# Autodesk Inventor assembly: Assembly1
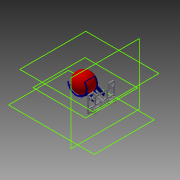
[picture p0: Inventor's stored thumbnail of the model, 180x180]
Saved by Autodesk Inventor 2014 (Build 180170000, 170)
## iProperties
Created: 2014-01-06
Part Number: Assembly1
Document SubType Name: Assembly
Designer: Tristan Debrunner
Author: Tristan Debrunner
## Documents named in this file (17)
- C:\Users\Tristan Debrunner\Documents\FRC 2014\Chassis\Assembly1.iam
- C:\Users\Tristan Debrunner\Documents\FRC 2014\Chassis\32 in bar.ipt
- C:\Users\Tristan Debrunner\Documents\FRC 2014\Chassis\21 in bar.ipt
- C:\Users\Tristan Debrunner\Documents\FRC 2014\Chassis\Corner.ipt
- C:\Users\Tristan Debrunner\Documents\FRC 2014\Chassis\8 in bar.ipt
- C:\Users\Tristan Debrunner\Documents\FRC 2014\Chassis\6 in bar.ipt
- C:\Users\Tristan Debrunner\Documents\FRC 2014\Chassis\Other corner.ipt
- C:\Users\Tristan Debrunner\Documents\FRC 2014\Chassis\2 hole plate.ipt
- C:\Users\Tristan Debrunner\Documents\Inventor\CIMple Box.iam
- C:\Users\Tristan Debrunner\Documents\FRC 2014\Claw Design\Inner.ipt
- C:\Users\Tristan Debrunner\Documents\FRC 2014\Claw Design\rod.ipt
- C:\Users\Tristan Debrunner\Documents\FRC 2014\Claw Design\Outer.ipt
- C:\Users\Tristan Debrunner\Documents\FRC 2014\Chassis\wheel.ipt
- C:\Users\Tristan Debrunner\Documents\FRC 2014\Chassis\Piston.iam
- C:\Users\Tristan Debrunner\Documents\FRC 2014\Chassis\5 in bar.ipt
- C:\Users\Tristan Debrunner\Documents\FRC 2014\Chassis\PG-71-am-0914.ipt
- C:\Users\Tristan Debrunner\Documents\FRC 2014\Chassis\ball.ipt
## Components (57 placed, 16 different names)
1. 32 in bar:1 — Mate:1, Mate:2, Angle:1, Mate:6, Mate:7, Mate:8, Mate:11, Mate:116, Mate:121
2. 21 in bar:1 — Mate:3, Mate:4, Angle:2, Angle:3, Mate:5, Mate:19, Mate:20, Mate:23, Mate:55, Mate:56, Mate:60, Mate:61, Mate:62, Mate:65
3. 21 in bar:2 — Mate:9, Mate:10, Mate:12, Mate:13, Mate:14, Mate:17, Mate:51, Mate:52, Mate:54, Mate:67, Mate:68, Mate:72, Angle:8
4. Corner:1 — Mate:1, Mate:2, Mate:3, Mate:4, Angle:1, Angle:2, Angle:3, Mate:5, Mate:6
5. Corner:2 — Mate:7, Mate:8, Mate:9, Mate:10, Mate:11, Mate:12
6. Corner:3 — Mate:19, Mate:20, Mate:21, Mate:22, Mate:23, Mate:24
7. Corner:4 — Mate:13, Mate:14, Mate:15, Mate:16, Mate:17, Mate:18
8. 6 in bar:1 — Mate:21, Mate:22, Mate:24, Mate:31, Mate:32, Mate:35
9. 6 in bar:2 — Mate:15, Mate:16, Mate:18, Mate:25, Mate:26, Mate:29, Flush:1
10. 6 in bar:3 — Mate:33, Mate:34, Mate:36, Mate:43, Mate:44, Mate:48
11. 6 in bar:4 — Mate:27, Mate:28, Mate:30, Mate:37, Mate:38, Mate:42
12. Corner:5 — Mate:25, Mate:26, Mate:27, Mate:28, Mate:29, Mate:30
13. Corner:6 — Mate:31, Mate:32, Mate:33, Mate:34, Mate:35, Mate:36
14. 32 in bar:2 — Mate:39, Mate:40, Mate:41, Mate:45, Mate:46, Mate:47, Mate:49, Mate:50, Mate:53, Mate:57, Mate:58, Mate:59, Mate:82, Mate:85, Mate:87, Mate:90, Mate:92, Mate:94, Mate:96
15. Corner:7 — Mate:37, Mate:38, Mate:39, Mate:40, Mate:41, Mate:42
16. Corner:8 — Mate:43, Mate:44, Mate:45, Mate:46, Mate:47, Mate:48
17. Corner:9 — Mate:49, Mate:50, Mate:51, Mate:52, Mate:53, Mate:54
18. Corner:10 — Mate:55, Mate:56, Mate:57, Mate:58, Mate:59, Mate:60
19. Corner:11 — Mate:61, Mate:62, Mate:63, Mate:64, Mate:65, Mate:66
20. 32 in bar:3 — Mate:63, Mate:64, Mate:66, Mate:69, Mate:70, Mate:71, Mate:73, Mate:76, Mate:77, Mate:79, Mate:81, Mate:98, Mate:100, Mate:102, Mate:117, Mate:118, Mate:122, Mate:123, Mate:129, Mate:130, Mate:131, Mate:132, Angle:6, Angle:7
21. Corner:12 — Mate:67, Mate:68, Mate:69, Mate:70, Mate:71, Mate:72
22. 8 in bar:1 — Mate:74, Mate:75, Mate:78, Mate:80, Mate:83, Mate:84, Mate:86, Mate:88, Mate:107, Mate:108, Mate:109
23. 8 in bar:2 — Mate:89, Mate:91, Mate:93, Mate:95, Mate:97, Mate:99, Mate:101, Mate:103, Mate:104, Mate:105, Mate:106
24. Other corner:1 — Mate:73, Mate:74, Mate:78
25. Other corner:2 — Mate:75, Mate:76, Mate:77
26. 2 hole plate:1 — Mate:79, Mate:80, Mate:81
27. Other corner:3 — Mate:82, Mate:83
28. Other corner:4 — Mate:84, Mate:85
29. 2 hole plate:2 — Mate:86, Mate:87, Mate:88
30. 2 hole plate:3 — Mate:89, Mate:90, Mate:92
31. 2 hole plate:4 — Mate:91, Mate:98, Mate:103
32. Other corner:5 — Mate:93, Mate:94
33. Other corner:6 — Mate:95, Mate:96, Mate:97
34. Other corner:7 — Mate:101, Mate:102
35. Other corner:8 — Mate:99, Mate:100
36. Corner:13 — Mate:104, Mate:105, Mate:106, Mate:110, Mate:111, Mate:112
37. Corner:14 — Mate:107, Mate:108, Mate:109, Mate:113, Mate:114, Mate:115
38. 8 in bar:3 — Mate:110, Mate:111, Mate:112, Mate:127
39. 8 in bar:4 — Mate:113, Mate:114, Mate:115, Mate:126, Mate:128
40. CIMple Box:1 [sub-assembly] — Mate:124, Mate:125, Angle:4, Insert:8
41. CIMple Box:2 [sub-assembly] — Mate:119, Mate:120, Angle:5, Insert:9
42. 6 in bar:5 — Mate:116, Mate:117, Mate:118, Mate:119, Mate:120, Angle:5
43. 6 in bar:6 — Mate:121, Mate:122, Mate:123, Mate:124, Mate:125, Angle:4
44. Inner:1 — Insert:1, Insert:2, Mate:128, Insert:3, Insert:4, Mate:135, Tangent:1
45. rod:1 — Insert:1, Mate:126
46. rod:2 — Insert:2, Mate:127
47. Outer:1 — Insert:5, Insert:6, Mate:134, Mate:135
48. rod:3 — Insert:3, Insert:5
49. rod:4 — Insert:4, Insert:6, Mate:134
50. wheel:1 — Insert:8
51. wheel:2 — Insert:9, Tangent:2
52. Piston:1 [sub-assembly] — Mate:133
53. 5 in bar:1 — Mate:129, Mate:132, Angle:7
54. 5 in bar:2 — Mate:130, Mate:131, Angle:6, Mate:133
55. PG-71-am-0914:1
56. PG-71-am-0914:2
57. ball:1 — Tangent:1
## Relationships (154: Mate 135, Angle 8, Insert 8, Tangent 2, Flush 1)
- Mate:1: 32 in bar:1 ↔ Corner:1
- Mate:2: 32 in bar:1 ↔ Corner:1
- Mate:3: 21 in bar:1 ↔ Corner:1
- Mate:4: 21 in bar:1 ↔ Corner:1
- Angle:1 (0 deg): 32 in bar:1 ↔ Corner:1
- Angle:2 (0 deg): 21 in bar:1 ↔ Corner:1
- Angle:3 (0 deg): 21 in bar:1 ↔ Corner:1
- Mate:5: 21 in bar:1 ↔ Corner:1
- Mate:6: 32 in bar:1 ↔ Corner:1
- Mate:7: 32 in bar:1 ↔ Corner:2
- Mate:8: 32 in bar:1 ↔ Corner:2
- Mate:9: 21 in bar:2 ↔ Corner:2
- Mate:10: 21 in bar:2 ↔ Corner:2
- Mate:11: 32 in bar:1 ↔ Corner:2
- Mate:12: 21 in bar:2 ↔ Corner:2
- Mate:13: 21 in bar:2 ↔ Corner:4
- Mate:14: 21 in bar:2 ↔ Corner:4
- Mate:15: Corner:4 ↔ 6 in bar:2
- Mate:16: Corner:4 ↔ 6 in bar:2
- Mate:17: 21 in bar:2 ↔ Corner:4
- Mate:18: Corner:4 ↔ 6 in bar:2
- Mate:19: 21 in bar:1 ↔ Corner:3
- Mate:20: 21 in bar:1 ↔ Corner:3
- Mate:21: Corner:3 ↔ 6 in bar:1
- Mate:22: Corner:3 ↔ 6 in bar:1
- Mate:23: 21 in bar:1 ↔ Corner:3
- Mate:24: Corner:3 ↔ 6 in bar:1
- Mate:25: 6 in bar:2 ↔ Corner:5
- Mate:26: 6 in bar:2 ↔ Corner:5
- Mate:27: 6 in bar:4 ↔ Corner:5
- Mate:28: 6 in bar:4 ↔ Corner:5
- Mate:29: 6 in bar:2 ↔ Corner:5
- Mate:30: 6 in bar:4 ↔ Corner:5
- Mate:31: 6 in bar:1 ↔ Corner:6
- Mate:32: 6 in bar:1 ↔ Corner:6
- Mate:33: 6 in bar:3 ↔ Corner:6
- Mate:34: 6 in bar:3 ↔ Corner:6
- Mate:35: 6 in bar:1 ↔ Corner:6
- Mate:36: 6 in bar:3 ↔ Corner:6
- Mate:37: 6 in bar:4 ↔ Corner:7
- Mate:38: 6 in bar:4 ↔ Corner:7
- Mate:39: 32 in bar:2 ↔ Corner:7
- Mate:40: 32 in bar:2 ↔ Corner:7
- Mate:41: 32 in bar:2 ↔ Corner:7
- Mate:42: 6 in bar:4 ↔ Corner:7
- Mate:43: 6 in bar:3 ↔ Corner:8
- Mate:44: 6 in bar:3 ↔ Corner:8
- Mate:45: 32 in bar:2 ↔ Corner:8
- Mate:46: 32 in bar:2 ↔ Corner:8
- Mate:47: 32 in bar:2 ↔ Corner:8
- Mate:48: 6 in bar:3 ↔ Corner:8
- Mate:49: 32 in bar:2 ↔ Corner:9
- Mate:50: 32 in bar:2 ↔ Corner:9
- Mate:51: 21 in bar:2 ↔ Corner:9
- Mate:52: 21 in bar:2 ↔ Corner:9
- Mate:53: 32 in bar:2 ↔ Corner:9
- Mate:54: 21 in bar:2 ↔ Corner:9
- Mate:55: 21 in bar:1 ↔ Corner:10
- Mate:56: 21 in bar:1 ↔ Corner:10
- Mate:57: 32 in bar:2 ↔ Corner:10
- Mate:58: 32 in bar:2 ↔ Corner:10
- Mate:59: 32 in bar:2 ↔ Corner:10
- Mate:60: 21 in bar:1 ↔ Corner:10
- Mate:61: 21 in bar:1 ↔ Corner:11
- Mate:62: 21 in bar:1 ↔ Corner:11
- Mate:63: Corner:11 ↔ 32 in bar:3
- Mate:64: Corner:11 ↔ 32 in bar:3
- Mate:65: 21 in bar:1 ↔ Corner:11
- Mate:66: Corner:11 ↔ 32 in bar:3
- Mate:67: 21 in bar:2 ↔ Corner:12
- Mate:68: 21 in bar:2 ↔ Corner:12
- Mate:69: 32 in bar:3 ↔ Corner:12
- Mate:70: 32 in bar:3 ↔ Corner:12
- Mate:71: 32 in bar:3 ↔ Corner:12
- Mate:72: 21 in bar:2 ↔ Corner:12
- Mate:73: 32 in bar:3 ↔ Other corner:1
- Mate:74: 8 in bar:1 ↔ Other corner:1
- Mate:75: 8 in bar:1 ↔ Other corner:2
- Mate:76: 32 in bar:3 ↔ Other corner:2
- Mate:77: 32 in bar:3 ↔ Other corner:2
- Mate:78: 8 in bar:1 ↔ Other corner:1
- Mate:79: 32 in bar:3 ↔ 2 hole plate:1
- Mate:80: 8 in bar:1 ↔ 2 hole plate:1
- Mate:81: 32 in bar:3 ↔ 2 hole plate:1
- Mate:82: 32 in bar:2 ↔ Other corner:3
- Mate:83: 8 in bar:1 ↔ Other corner:3
- Mate:84: 8 in bar:1 ↔ Other corner:4
- Mate:85: 32 in bar:2 ↔ Other corner:4
- Mate:86: 8 in bar:1 ↔ 2 hole plate:2
- Mate:87: 32 in bar:2 ↔ 2 hole plate:2
- Mate:88: 8 in bar:1 ↔ 2 hole plate:2
- Mate:89: 8 in bar:2 ↔ 2 hole plate:3
- Mate:90: 32 in bar:2 ↔ 2 hole plate:3
- Mate:91: 8 in bar:2 ↔ 2 hole plate:4
- Mate:92: 32 in bar:2 ↔ 2 hole plate:3
- Mate:93: 8 in bar:2 ↔ Other corner:5
- Mate:94: 32 in bar:2 ↔ Other corner:5
- Mate:95: 8 in bar:2 ↔ Other corner:6
- Mate:96: 32 in bar:2 ↔ Other corner:6
- Mate:97: 8 in bar:2 ↔ Other corner:6
- Mate:98: 32 in bar:3 ↔ 2 hole plate:4
- Mate:99: 8 in bar:2 ↔ Other corner:8
- Mate:100: 32 in bar:3 ↔ Other corner:8
- Mate:101: 8 in bar:2 ↔ Other corner:7
- Mate:102: 32 in bar:3 ↔ Other corner:7
- Mate:103: 8 in bar:2 ↔ 2 hole plate:4
- Mate:104: 8 in bar:2 ↔ Corner:13
- Mate:105: 8 in bar:2 ↔ Corner:13
- Mate:106: 8 in bar:2 ↔ Corner:13
- Mate:107: 8 in bar:1 ↔ Corner:14
- Mate:108: 8 in bar:1 ↔ Corner:14
- Mate:109: 8 in bar:1 ↔ Corner:14
- Mate:110: Corner:13 ↔ 8 in bar:3
- Mate:111: Corner:13 ↔ 8 in bar:3
- Mate:112: Corner:13 ↔ 8 in bar:3
- Mate:113: Corner:14 ↔ 8 in bar:4
- Mate:114: Corner:14 ↔ 8 in bar:4
- Mate:115: Corner:14 ↔ 8 in bar:4
- Mate:116: 32 in bar:1 ↔ 6 in bar:5
- Mate:117: 32 in bar:3 ↔ 6 in bar:5
- Mate:118: 32 in bar:3 ↔ 6 in bar:5
- Mate:119: CIMple Box:2 ↔ 6 in bar:5
- Mate:120: CIMple Box:2 ↔ 6 in bar:5
- Mate:121: 32 in bar:1 ↔ 6 in bar:6
- Mate:122: 32 in bar:3 ↔ 6 in bar:6
- Mate:123: 32 in bar:3 ↔ 6 in bar:6
- Mate:124: CIMple Box:1 ↔ 6 in bar:6
- Mate:125: CIMple Box:1 ↔ 6 in bar:6
- Angle:4 (180 deg): CIMple Box:1 ↔ 6 in bar:6
- Angle:5 (0 deg): CIMple Box:2 ↔ 6 in bar:5
- Insert:1: Inner:1 ↔ rod:1
- Insert:2: Inner:1 ↔ rod:2
- Mate:126: 8 in bar:4 ↔ rod:1
- Mate:127: 8 in bar:3 ↔ rod:2
- Mate:128: 8 in bar:4 ↔ Inner:1
- Insert:3: Inner:1 ↔ rod:3
- Insert:4: Inner:1 ↔ rod:4
- Insert:5: Outer:1 ↔ rod:3
- Insert:6: Outer:1 ↔ rod:4
- Insert:8: CIMple Box:1 ↔ wheel:1
- Insert:9: CIMple Box:2 ↔ wheel:2
- Mate:129: 32 in bar:3 ↔ 5 in bar:1
- Mate:130: 32 in bar:3 ↔ 5 in bar:2
- Mate:131: 32 in bar:3 ↔ 5 in bar:2
- Mate:132: 32 in bar:3 ↔ 5 in bar:1
- Angle:6 (180 deg): 32 in bar:3 ↔ 5 in bar:2
- Angle:7 (180 deg): 32 in bar:3 ↔ 5 in bar:1
- Mate:133: Piston:1 ↔ 5 in bar:2
- Mate:134: Outer:1 ↔ rod:4
- Mate:135: Inner:1 ↔ Outer:1
- Tangent:1: Inner:1 ↔ ball:1
- Angle:8 (0 deg): 21 in bar:2
- Tangent:2: wheel:2
- Flush:1 (508 mm): 6 in bar:2
